# Autodesk Inventor assembly: Cameramounting
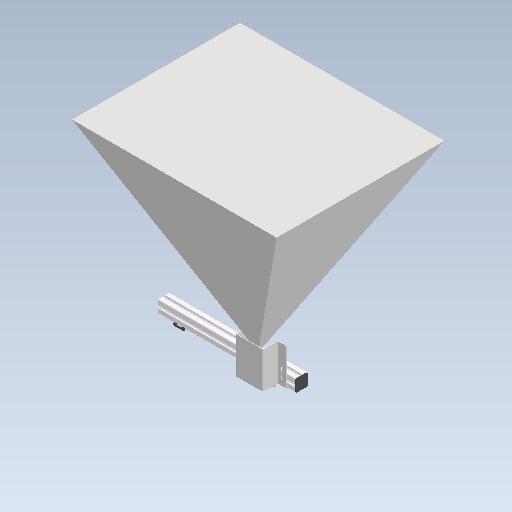
[picture p0: Inventor's stored thumbnail of the model, 512x512]
Saved by Autodesk Inventor 2020 (Build 240168000, 168)
## iProperties
Created: 2019-11-06
Part Number: Cameramounting
Document SubType Name: Assembly
Designer: nicoc
Author: nicoc
## Documents named in this file (9)
- D:\Repos\P5-AIonFPGA\cad\Cameramounting\Cameramounting.iam
- D:\Repos\P5-AIonFPGA\cad\Cameramounting\Camera\11165907_VCXU-13C.iam
- D:\Repos\P5-AIonFPGA\cad\Cameramounting\MountingAdapter.ipt
- D:\Repos\P5-AIonFPGA\cad\Cameramounting\Lense.ipt
- D:\Repos\P5-AIonFPGA\cad\Cameramounting\CameraProtection.ipt
- D:\Repos\P5-AIonFPGA\cad\Cameramounting\item_7000009_Profile_8_40x40_E_L=450.ipt
- D:\Repos\P5-AIonFPGA\cad\Cameramounting\FieldofView.ipt
- D:\Repos\P5-AIonFPGA\cad\Cameramounting\item_0002601_Cap_8_40x40_2.ipt
- D:\Repos\P5-AIonFPGA\cad\BasicFramework\UniversalHolder\item_0062790_Universal_Holder_with_Securing_Strap_8_180_1.iam
## Components (8 placed, 8 different names)
1. 11165907_VCXU-13C:1 [sub-assembly] — Mate:1, Mate:2, Mate:3, Flush:1, Mate:5, Insert:1, Flush:5, Mate:8, Mate:9
2. MountingAdapter:1 — Mate:1, Mate:2, Mate:3, Mate:4, Mate:7
3. Lense:1 — Mate:5, Insert:1, Flush:6
4. CameraProtection:1 — Mate:6, Flush:3, Mate:7
5. item_7000009_Profile_8_40x40_E_L=450:1 — Mate:4, Flush:1, Mate:6, Flush:3, Flush:5, Mate:10, Flush:7, Flush:8, Mate:11, Flush:9, Flush:10
6. FieldofView:1 — Flush:6, Mate:8, Mate:9
7. item_0002601_Cap_8_40x40_2:1 — Mate:10, Flush:7, Flush:8
8. item_0062790_Universal_Holder_with_Securing_Strap_8_180_1:1 [sub-assembly] — Mate:11, Flush:9, Flush:10
## Relationships (20: Mate 11, Flush 8, Insert 1)
- Mate:1: 11165907_VCXU-13C:1 ↔ MountingAdapter:1
- Mate:2: 11165907_VCXU-13C:1 ↔ MountingAdapter:1
- Mate:3: 11165907_VCXU-13C:1 ↔ MountingAdapter:1
- Mate:4: MountingAdapter:1 ↔ item_7000009_Profile_8_40x40_E_L=450:1
- Flush:1 (335.65 mm): 11165907_VCXU-13C:1 ↔ item_7000009_Profile_8_40x40_E_L=450:1
- Mate:5: 11165907_VCXU-13C:1 ↔ Lense:1
- Insert:1: 11165907_VCXU-13C:1 ↔ Lense:1
- Mate:6: CameraProtection:1 ↔ item_7000009_Profile_8_40x40_E_L=450:1
- Flush:3: CameraProtection:1 ↔ item_7000009_Profile_8_40x40_E_L=450:1
- Flush:5 (-7.2 mm): 11165907_VCXU-13C:1 ↔ item_7000009_Profile_8_40x40_E_L=450:1
- Mate:7 (3 mm): MountingAdapter:1 ↔ CameraProtection:1
- Flush:6 (630 mm): Lense:1 ↔ FieldofView:1
- Mate:8 (-19.35 mm): 11165907_VCXU-13C:1 ↔ FieldofView:1
- Mate:9 (-19.5 mm): 11165907_VCXU-13C:1 ↔ FieldofView:1
- Mate:10: item_7000009_Profile_8_40x40_E_L=450:1 ↔ item_0002601_Cap_8_40x40_2:1
- Flush:7: item_7000009_Profile_8_40x40_E_L=450:1 ↔ item_0002601_Cap_8_40x40_2:1
- Flush:8: item_7000009_Profile_8_40x40_E_L=450:1 ↔ item_0002601_Cap_8_40x40_2:1
- Mate:11: item_7000009_Profile_8_40x40_E_L=450:1 ↔ item_0062790_Universal_Holder_with_Securing_Strap_8_180_1:1
- Flush:9 (10 mm): item_7000009_Profile_8_40x40_E_L=450:1 ↔ item_0062790_Universal_Holder_with_Securing_Strap_8_180_1:1
- Flush:10 (50 mm): item_7000009_Profile_8_40x40_E_L=450:1 ↔ item_0062790_Universal_Holder_with_Securing_Strap_8_180_1:1
